# Autodesk Inventor assembly: DriveTrain
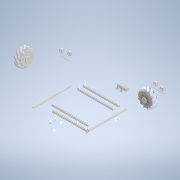
[picture p0: Inventor's stored thumbnail of the model, 180x180]
Saved by Autodesk Inventor 2020.2 (Build 242310000, 310)
## iProperties
Created: 2020-01-29
Part Number: DriveTrain
Document SubType Name: Assembly
Designer: yukin
Author: yukin
## Documents named in this file (14)
- C:\Autodesk\Files\CAD\Robotics 2019-2020\Assembly\DriveTrain\DriveTrain.iam
- C:\Autodesk\Files\CAD\Robotics 2019-2020\Assembly\DriveTrain\RevHexMotor\RevHexMotor.iam
- C:\Autodesk\Files\CAD\Robotics 2019-2020\Assembly\DriveTrain\MotorMount_vCAD.ipt
- C:\Autodesk\Files\CAD\Robotics 2019-2020\Assembly\DriveTrain\Extrusions\17in.ipt
- C:\Autodesk\Files\CAD\Robotics 2019-2020\Assembly\DriveTrain\CornerBracket.ipt
- C:\Autodesk\Files\CAD\Robotics 2019-2020\Assembly\DriveTrain\MotorMountBackSide.ipt
- C:\Autodesk\Files\CAD\Robotics 2019-2020\Assembly\DriveTrain\Extrusions\18in.ipt
- C:\Autodesk\Files\CAD\Robotics 2019-2020\Assembly\DriveTrain\BearingHolder.ipt
- C:\Autodesk\Files\CAD\Robotics 2019-2020\Assembly\DriveTrain\LMecaWheel\LMecaWheel.iam
- C:\Autodesk\Files\CAD\Robotics 2019-2020\Assembly\DriveTrain\RMecaWheel\RMecaWheel.iam
- C:\Autodesk\Files\CAD\Robotics 2019-2020\Assembly\DriveTrain\HexHub.ipt
- C:\Autodesk\Files\CAD\Robotics 2019-2020\Assembly\DriveTrain\WheelMount_v1_vCAD.ipt
- C:\Autodesk\Files\CAD\Robotics 2019-2020\Assembly\DriveTrain\WheelMount_v2_vCAD.ipt
- C:\Autodesk\Files\CAD\Robotics 2019-2020\Assembly\DriveTrain\HexShaft.ipt
## Components (39 placed, 13 different names)
1. RevHexMotor:1 [sub-assembly] — Rotational:1, Insert:1
2. MotorMount_vCAD:1 — Rotational:1, Flush:21
3. 17in:1 — Flush:12, Flush:13, Mate:7, Mate:8, Flush:14, Flush:15
4. 17in:2 — Flush:8, Flush:9, Mate:5, Flush:10, Mate:6, Flush:11
5. CornerBracket:1
6. CornerBracket:2
7. CornerBracket:3 — Mate:8, Flush:14, Flush:15
8. CornerBracket:4 — Flush:12, Flush:13, Mate:7
9. CornerBracket:5 — Flush:8, Flush:9, Mate:5
10. CornerBracket:6 — Flush:10, Mate:6, Flush:11
11. CornerBracket:7
12. CornerBracket:8
13. MotorMountBackSide:1 — Insert:1, Flush:21
14. 18in:1
15. 18in:2 — Flush:37, Flush:47, Flush:48, Mate:30
16. CornerBracket:9
17. CornerBracket:10 — Flush:47, Flush:48, Mate:29, Flush:50, Flush:51, Mate:30
18. CornerBracket:11
19. CornerBracket:12
20. 17in:3 — Flush:39, Flush:40, Mate:24, Flush:43, Flush:44, Mate:26, Mate:29, Flush:49, Flush:50, Flush:51
21. 17in:4 — Flush:37, Mate:25, Flush:41, Flush:42, Flush:45, Flush:46, Mate:27
22. CornerBracket:13 — Flush:39, Flush:40, Mate:24, Flush:49
23. CornerBracket:14 — Flush:43, Flush:44, Mate:26
24. CornerBracket:15 — Mate:25, Flush:41, Flush:42
25. CornerBracket:16 — Flush:45, Flush:46, Mate:27
26. BearingHolder:1
27. BearingHolder:2
28. BearingHolder:3
29. BearingHolder:4
30. LMecaWheel:2 [sub-assembly] — Insert:10, Insert:11, Insert:12, Insert:13
31. RMecaWheel:1 [sub-assembly] — Insert:2, Insert:3, Insert:6, Insert:7
32. HexHub:2 — Insert:8, Insert:9
33. HexHub:3 — Insert:4, Insert:5
34. WheelMount_v1_vCAD:1 — Insert:12, Insert:13
35. WheelMount_v1_vCAD:2 — Insert:6, Insert:7
36. WheelMount_v2_vCAD:1 — Insert:2, Insert:3, Insert:4, Insert:5
37. HexShaft:1
38. HexShaft:2
39. WheelMount_v2_vCAD:2 — Insert:8, Insert:9, Insert:10, Insert:11
## Relationships (47: Flush 23, Insert 13, Mate 10, RevoluteJoint 1)
- Rotational:1 [RevoluteJoint]: RevHexMotor:1 ↔ MotorMount_vCAD:1
- Flush:8: 17in:2 ↔ CornerBracket:5
- Flush:9: 17in:2 ↔ CornerBracket:5
- Mate:5: 17in:2 ↔ CornerBracket:5
- Flush:10: 17in:2 ↔ CornerBracket:6
- Mate:6: 17in:2 ↔ CornerBracket:6
- Flush:11: 17in:2 ↔ CornerBracket:6
- Flush:12: 17in:1 ↔ CornerBracket:4
- Flush:13: 17in:1 ↔ CornerBracket:4
- Mate:7: 17in:1 ↔ CornerBracket:4
- Mate:8: 17in:1 ↔ CornerBracket:3
- Flush:14: 17in:1 ↔ CornerBracket:3
- Flush:15: 17in:1 ↔ CornerBracket:3
- Insert:1: RevHexMotor:1 ↔ MotorMountBackSide:1
- Flush:21: MotorMount_vCAD:1 ↔ MotorMountBackSide:1
- Flush:37: 18in:2 ↔ 17in:4
- Flush:39: 17in:3 ↔ CornerBracket:13
- Flush:40: 17in:3 ↔ CornerBracket:13
- Mate:24: 17in:3 ↔ CornerBracket:13
- Mate:25: 17in:4 ↔ CornerBracket:15
- Flush:41: 17in:4 ↔ CornerBracket:15
- Flush:42: 17in:4 ↔ CornerBracket:15
- Flush:43: 17in:3 ↔ CornerBracket:14
- Flush:44: 17in:3 ↔ CornerBracket:14
- Mate:26: 17in:3 ↔ CornerBracket:14
- Flush:45: 17in:4 ↔ CornerBracket:16
- Flush:46: 17in:4 ↔ CornerBracket:16
- Mate:27: 17in:4 ↔ CornerBracket:16
- Insert:2: RMecaWheel:1 ↔ WheelMount_v2_vCAD:1
- Insert:3: RMecaWheel:1 ↔ WheelMount_v2_vCAD:1
- Insert:4: HexHub:3 ↔ WheelMount_v2_vCAD:1
- Insert:5: HexHub:3 ↔ WheelMount_v2_vCAD:1
- Insert:6: RMecaWheel:1 ↔ WheelMount_v1_vCAD:2
- Insert:7: RMecaWheel:1 ↔ WheelMount_v1_vCAD:2
- Insert:8: HexHub:2 ↔ WheelMount_v2_vCAD:2
- Insert:9: HexHub:2 ↔ WheelMount_v2_vCAD:2
- Insert:10: LMecaWheel:2 ↔ WheelMount_v2_vCAD:2
- Insert:11: LMecaWheel:2 ↔ WheelMount_v2_vCAD:2
- Insert:12: LMecaWheel:2 ↔ WheelMount_v1_vCAD:1
- Insert:13: LMecaWheel:2 ↔ WheelMount_v1_vCAD:1
- Flush:47: 18in:2 ↔ CornerBracket:10
- Flush:48 (0.3556 mm): 18in:2 ↔ CornerBracket:10
- Mate:29: CornerBracket:10 ↔ 17in:3
- Flush:49: 17in:3 ↔ CornerBracket:13
- Flush:50: CornerBracket:10 ↔ 17in:3
- Flush:51: CornerBracket:10 ↔ 17in:3
- Mate:30: 18in:2 ↔ CornerBracket:10
